# Autodesk Inventor assembly: Buffer
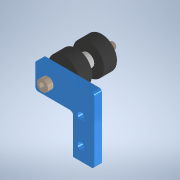
[picture p0: Inventor's stored thumbnail of the model, 180x180]
Saved by Autodesk Inventor 2021 (Build 250183000, 183)
## iProperties
Created: 2021-09-25
Part Number: Buffer
Document SubType Name: Assembly
Designer: Jorian Brusind
Author: Jorian Brusind
## Documents named in this file (7)
- C:\Users\Jorian Brusind\Documents\GitHub\HyperRail\Inventor Files\Buffer.iam
- C:\Users\Jorian Brusind\Documents\GitHub\HyperRail\Inventor Files\Buffer_Mount.ipt
- C:\Users\Jorian Brusind\Documents\GitHub\HyperRail\Inventor Files\11mm_BearingWheel.ipt
- C:\Users\Jorian Brusind\Documents\GitHub\HyperRail\Inventor Files\Metric bolt\Bolt M5 50mm.ipt
- C:\Users\Jorian Brusind\Documents\GitHub\HyperRail\Inventor Files\5mm_Spacer.ipt
- C:\Users\Jorian Brusind\Documents\GitHub\HyperRail\Inventor Files\8mm_Spacer.ipt
- C:\Users\Jorian Brusind\Documents\GitHub\PersonalProjects\HyperRail\Inventor Files\Metric nuts\Nut M5.ipt
## Components (7 placed, 6 different names)
1. Buffer_Mount:1 — Mate:5, Mate:7, Mate:10, Mate:14
2. 11mm_BearingWheel:1 — Mate:8, Mate:15, Mate:17
3. 11mm_BearingWheel:2 — Mate:5, Mate:9, Mate:13
4. Bolt M5 50mm:1 — Mate:7, Mate:8, Mate:9, Mate:10, Mate:11, Mate:12, Mate:16
5. 5mm_Spacer:1 — Mate:11, Mate:14
6. 8mm_Spacer:1 — Mate:12, Mate:13, Mate:15
7. Nut M5:1 — Mate:16, Mate:17
## Relationships (12: Mate 12)
- Mate:5 (5 mm): Buffer_Mount:1 ↔ 11mm_BearingWheel:2
- Mate:7: Buffer_Mount:1 ↔ Bolt M5 50mm:1
- Mate:8: 11mm_BearingWheel:1 ↔ Bolt M5 50mm:1
- Mate:9: 11mm_BearingWheel:2 ↔ Bolt M5 50mm:1
- Mate:10: Buffer_Mount:1 ↔ Bolt M5 50mm:1
- Mate:11: Bolt M5 50mm:1 ↔ 5mm_Spacer:1
- Mate:12: Bolt M5 50mm:1 ↔ 8mm_Spacer:1
- Mate:13: 11mm_BearingWheel:2 ↔ 8mm_Spacer:1
- Mate:14: Buffer_Mount:1 ↔ 5mm_Spacer:1
- Mate:15: 11mm_BearingWheel:1 ↔ 8mm_Spacer:1
- Mate:16: Bolt M5 50mm:1 ↔ Nut M5:1
- Mate:17: 11mm_BearingWheel:1 ↔ Nut M5:1
